# Autodesk Inventor assembly: Connect
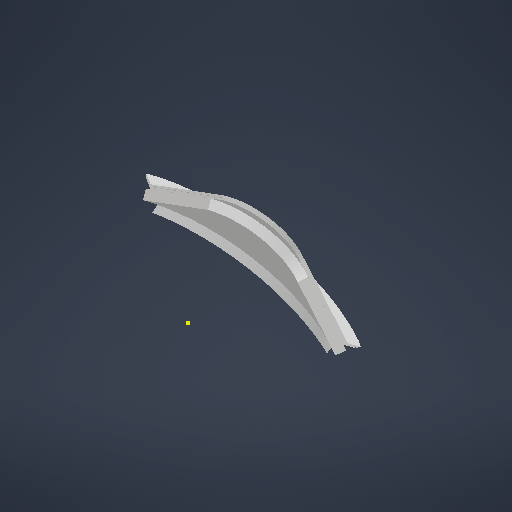
[picture p0: Inventor's stored thumbnail of the model, 512x512]
Saved by Autodesk Inventor 2026.2 (Build 302298000, 298)
## iProperties
Created: 2025-12-16
Part Number: Connect
Document SubType Name: Assembly
Designer: Thoma
Author: Thoma
## Documents named in this file (3)
- C:\Users\Thoma\OneDrive\Desktop\Inventor\Quarter_Open\Version_2_Cone\Connect.iam
- C:\Users\Thoma\OneDrive\Desktop\Inventor\Quarter_Open\Version_2_Cone\Cover_Upper_v2.ipt
- C:\Users\Thoma\OneDrive\Desktop\Inventor\Quarter_Open\Version_2_Cone\rod.ipt
## Components (2 placed, 2 different names)
1. Cover_Upper_v2:2 — Mate:14, Flush:2
2. rod:1 — Mate:14, Flush:2
## Relationships (2: Mate 1, Flush 1)
- Mate:14: Cover_Upper_v2:2 ↔ rod:1
- Flush:2 (17.4 mm): Cover_Upper_v2:2 ↔ rod:1
